# Autodesk Inventor assembly: Limit Switch KW12-3
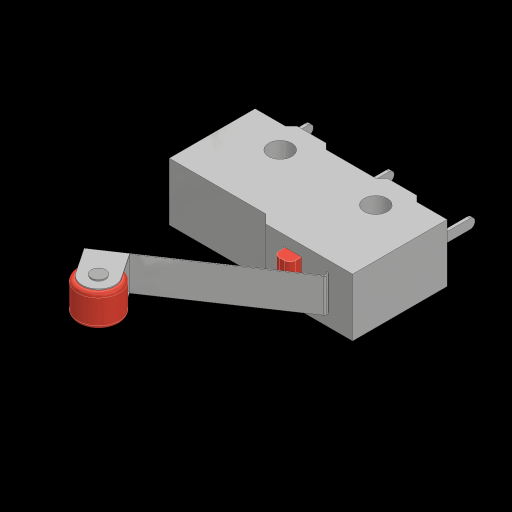
[picture p0: Inventor's stored thumbnail of the model, 512x512]
Saved by Autodesk Inventor 2023 (Build 270158000, 158)
## iProperties
Created: 2023-08-04
Part Number: Limit Switch KW12-3
Document SubType Name: Assembly
Designer: tandu
Author: tandu
## iProperties of the stored document Nc.ipt
Created: 2023-08-04
Part Number: Nc
Material: Steel
Document SubType Name: Modeling
Designer: tandu
Density: 7.85 g/cm^3
Appearance: Default
Author: tandu
## iProperties of the stored document haste.ipt
Created: 2023-08-04
Part Number: haste
Material: Steel
Document SubType Name: Modeling
Designer: tandu
Density: 7.85 g/cm^3
Appearance: Default
Author: tandu
## iProperties of the stored document Fim de Curso - KW12-3.iam
Created: 2020-05-19
Part Number: Fim de Curso - KW12-3
Document SubType Name: Assembly
Designer: tandu
Sending System: Autodesk Translation Framework v9.3.0.1241
Preprocessor: ST-DEVELOPER v18.1
Title: c:\worker\convert-fusion-r04\tmp\job-1\1339\output\files\434cfe47-db58-40e9-b348-48f3873ac6f4\ff005539-6c8e-4882-8ede-d92c0df456a6.stp
## iProperties of the stored document Roldana.ipt
Created: 2023-08-04
Part Number: Roldana
Material: Steel
Document SubType Name: Modeling
Designer: tandu
Density: 7.85 g/cm^3
Appearance: Default
Author: tandu
## iProperties of the stored document No.ipt
Created: 2023-08-04
Part Number: No
Material: Steel
Document SubType Name: Modeling
Designer: tandu
Density: 7.85 g/cm^3
Appearance: Default
Author: tandu
## iProperties of the stored document C.ipt
Created: 2023-08-04
Part Number: C
Material: Steel
Document SubType Name: Modeling
Designer: tandu
Density: 7.85 g/cm^3
Appearance: Default
Author: tandu
## iProperties of the stored document Botão.ipt
Created: 2023-08-04
Part Number: Botão
Material: Steel
Document SubType Name: Modeling
Designer: tandu
Density: 7.85 g/cm^3
Appearance: Default
Author: tandu
## iProperties of the stored document Eixo.ipt
Created: 2023-08-04
Part Number: Eixo
Material: Steel
Document SubType Name: Modeling
Designer: tandu
Density: 7.85 g/cm^3
Appearance: Default
Author: tandu
## iProperties of the stored document Corpo.ipt
Created: 2023-08-04
Part Number: Corpo
Material: Steel
Document SubType Name: Modeling
Designer: tandu
Density: 7.85 g/cm^3
Appearance: Default
Author: tandu
## Documents named in this file (11)
- C:\Users\tandu\Documents\GrabCAD\Robotic Arm Project\IndustrialStyledVersion\V1\Limit Switch KW12-3.iam
- **C:\Users\tandu\Documents\GrabCAD\Robotic Arm Project\IndustrialStyledVersion\V1\Limit Switch KW12-3.iam*LocalDocs*xAaaaa2daAaaaaaaaAaaaar1cZe*Fim de Curso - KW12-3.iam
- C:\Users\tandu\Documents\GrabCAD\Robotic Arm Project\IndustrialStyledVersion\V1\References\Fim de Curso - KW12-3.stp
- **C:\Users\tandu\Documents\GrabCAD\Robotic Arm Project\IndustrialStyledVersion\V1\Limit Switch KW12-3.iam*LocalDocs*xAaaaafcaAaaaaaaaAaaaarxiCd*Nc.ipt
- **C:\Users\tandu\Documents\GrabCAD\Robotic Arm Project\IndustrialStyledVersion\V1\Limit Switch KW12-3.iam*LocalDocs*xAaaaa4baAaaaaaaaAaaaahcwIg*haste.ipt
- **C:\Users\tandu\Documents\GrabCAD\Robotic Arm Project\IndustrialStyledVersion\V1\Limit Switch KW12-3.iam*LocalDocs*xAaaaqxdaAaaaaaaaAaaaa35t4a*Corpo.ipt
- **C:\Users\tandu\Documents\GrabCAD\Robotic Arm Project\IndustrialStyledVersion\V1\Limit Switch KW12-3.iam*LocalDocs*xAaaaqccaAaaaaaaaAaaaqryv4g*No.ipt
- **C:\Users\tandu\Documents\GrabCAD\Robotic Arm Project\IndustrialStyledVersion\V1\Limit Switch KW12-3.iam*LocalDocs*xAaaaamdaAaaaaaaaAaaaqz5dYc*C.ipt
- **C:\Users\tandu\Documents\GrabCAD\Robotic Arm Project\IndustrialStyledVersion\V1\Limit Switch KW12-3.iam*LocalDocs*xAaaaabcaAaaaaaaaAaaaahvxYc*Roldana.ipt
- **C:\Users\tandu\Documents\GrabCAD\Robotic Arm Project\IndustrialStyledVersion\V1\Limit Switch KW12-3.iam*LocalDocs*xAaaaqwdaAaaaaaaaAaaaavqiSh*Botão.ipt
- **C:\Users\tandu\Documents\GrabCAD\Robotic Arm Project\IndustrialStyledVersion\V1\Limit Switch KW12-3.iam*LocalDocs*xAaaaqfbaAaaaaaaaAaaaaostQd*Eixo.ipt
## Components (1 placed, 1 different names)
1. Fim de Curso - KW12-3:1 [sub-assembly] — Mate:1, Angle:1
## Relationships (2: Mate 1, Angle 1)
- Mate:1: Fim de Curso - KW12-3:1
- Angle:1 (0 deg): Fim de Curso - KW12-3:1
